# Autodesk Inventor assembly: NRF24L01L+Antenna
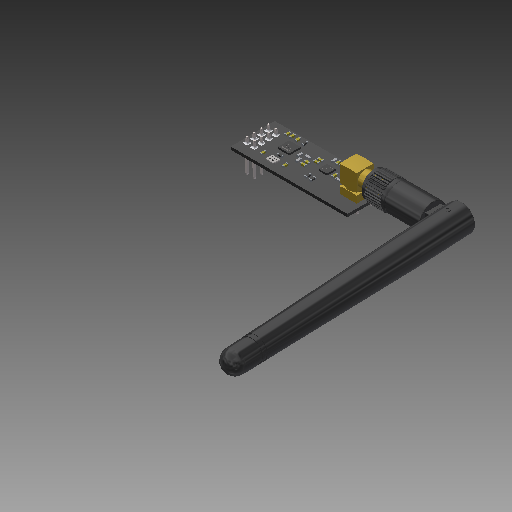
[picture p0: Inventor's stored thumbnail of the model, 512x512]
Saved by Autodesk Inventor 2019 (Build 230136000, 136)
## iProperties
Created: 2019-01-18
Part Number: NRF24L01L+Antenna
Document SubType Name: Assembly
Designer: Pulag
Sending System: SolidWorks 2016
Last Author: Condor
Last Saved: 2019-01-20
Author: Pulag
## Documents named in this file (3)
- C:\Users\Pulag\Documents\GitHub\24th_TDK_Project_D5\CAD\CAD file\nrf24l01p-pa-lna-1.snapshot.2\NRF24L01L + Antenna 2.4 GHz\NRF24L01L+Antenna.iam
- C:\Users\Pulag\Documents\GitHub\24th_TDK_Project_D5\CAD\CAD file\nrf24l01p-pa-lna-1.snapshot.2\NRF24L01L + Antenna 2.4 GHz\NRF24L01L.ipt
- C:\Users\Pulag\Documents\GitHub\24th_TDK_Project_D5\CAD\CAD file\nrf24l01p-pa-lna-1.snapshot.2\NRF24L01L + Antenna 2.4 GHz\Antenna assy.iam
## Components (2 placed, 2 different names)
1. NRF24L01L:1 — Mate:1, Flush:1
2. Antenna assy:1 [sub-assembly] — Mate:1, Flush:1
## Relationships (2: Mate 1, Flush 1)
- Mate:1: NRF24L01L:1 ↔ Antenna assy:1
- Flush:1: NRF24L01L:1 ↔ Antenna assy:1
